# Autodesk Inventor assembly: VersaPlanetary_Lite_0_Stage_3_8_Hex
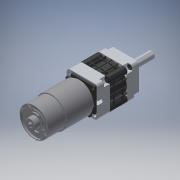
[picture p0: Inventor's stored thumbnail of the model, 180x180]
Saved by Autodesk Inventor 2019 (Build 230136000, 136)
## iProperties
Created: 2017-12-05
Part Number: VersaPlanetary_Lite_0_Stage_3_8_Hex
Description: STEP AP214
Document SubType Name: Assembly
Designer: leadere
Mass: 625.957 g
Surface Area: 744.288 cm^2
Volume: 153.893 cm^3
Density: 4.06749 g/cm^3
Sending System: SolidWorks 2017
Preprocessor: SwSTEP 2.0
Title: VersaPlanetary-Lite-0-Stage-NeveRest-20171205.STEP
Revision Number: ANY
## Documents named in this file (8)
- C:\Users\leadere\Documents\GrabCAD\2019 Robot\Imported Components\Gearboxes\VersaPlanetary Lite\VersaPlanetary_Lite_2_Stage_3_8_Hex_775.iam
- C:\Users\leadere\Documents\GrabCAD\2019 Robot\Imported Components\Gearboxes\VersaPlanetary Lite\VersaPlanetary Output Blocks_VP Lite Output Block.iam
- C:\Users\leadere\Documents\GrabCAD\2019 Robot\Imported Components\Gearboxes\VersaPlanetary Lite\VersaPlanetary Output Shafts_0.375_ Hex (217-2625-021).iam
- C:\Users\leadere\Documents\GrabCAD\2019 Robot\Imported Components\Gearboxes\VersaPlanetary Lite\217-2625-018 Rev1_98541A410.ipt
- C:\Users\leadere\Documents\GrabCAD\2019 Robot\Imported Components\Gearboxes\VersaPlanetary Lite\VersaPlanetary Input Blocks_VP LIte Input Block.iam
- C:\Users\leadere\Documents\GrabCAD\2019 Robot\Imported Components\Gearboxes\VersaPlanetary Lite\VersaPlanetary_Lite_Ring_Gear.ipt
- C:\Users\leadere\Documents\GrabCAD\2019 Robot\Imported Components\Gearboxes\VersaPlanetary Lite\217-2822-001 Rev4.ipt
- C:\Users\leadere\Documents\GrabCAD\2019 Robot\Imported Components\Motors\775pro.ipt
## Components (8 placed, 7 different names)
1. VersaPlanetary Output Blocks_VP Lite Output Block_1 [sub-assembly] — Mate:1, Mate:2
2. VersaPlanetary Output Shafts_0.375" Hex (217-2625-021)_2 [sub-assembly]
3. 217-2625-018 Rev1_98541A410_3
4. VersaPlanetary Input Blocks_VP LIte Input Block_4 [sub-assembly] — Mate:6, Mate:7, Mate:8, Mate:9
5. VersaPlanetary_Lite_Ring_Gear:1 — Mate:1, Mate:2, Mate:3, Mate:4, Mate:5
6. VersaPlanetary_Lite_Ring_Gear:2 — Mate:3, Mate:4, Mate:5, Mate:6, Mate:7
7. 217-2822-001 Rev4:1 — Mate:8, Mate:9, Mate:10, Mate:11
8. 775pro:1 — Mate:10, Mate:11
## Relationships (11: Mate 11)
- Mate:1: VersaPlanetary Output Blocks_VP Lite Output Block_1 ↔ VersaPlanetary_Lite_Ring_Gear:1
- Mate:2: VersaPlanetary Output Blocks_VP Lite Output Block_1 ↔ VersaPlanetary_Lite_Ring_Gear:1
- Mate:3: VersaPlanetary_Lite_Ring_Gear:1 ↔ VersaPlanetary_Lite_Ring_Gear:2
- Mate:4: VersaPlanetary_Lite_Ring_Gear:1 ↔ VersaPlanetary_Lite_Ring_Gear:2
- Mate:5: VersaPlanetary_Lite_Ring_Gear:1 ↔ VersaPlanetary_Lite_Ring_Gear:2
- Mate:6: VersaPlanetary Input Blocks_VP LIte Input Block_4 ↔ VersaPlanetary_Lite_Ring_Gear:2
- Mate:7: VersaPlanetary Input Blocks_VP LIte Input Block_4 ↔ VersaPlanetary_Lite_Ring_Gear:2
- Mate:8: VersaPlanetary Input Blocks_VP LIte Input Block_4 ↔ 217-2822-001 Rev4:1
- Mate:9: VersaPlanetary Input Blocks_VP LIte Input Block_4 ↔ 217-2822-001 Rev4:1
- Mate:10: 217-2822-001 Rev4:1 ↔ 775pro:1
- Mate:11: 217-2822-001 Rev4:1 ↔ 775pro:1
